# Autodesk Inventor assembly: Ensamblaje1
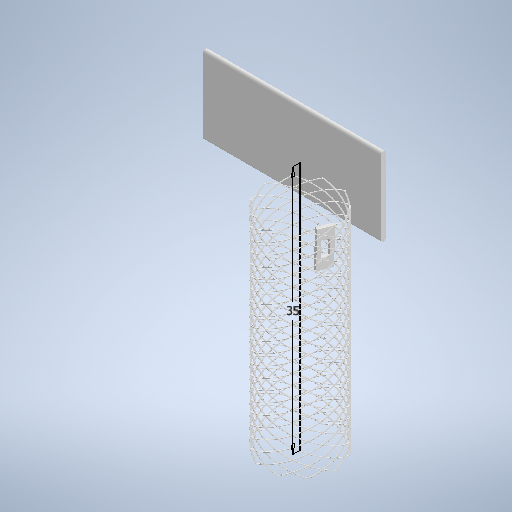
[picture p0: Inventor's stored thumbnail of the model, 512x512]
Saved by Autodesk Inventor 2025.2 (Build 292293000, 293)
## iProperties
Created: 2025-03-06
Part Number: Ensamblaje1
Document SubType Name: Assembly
Designer: julia
Author: julia
## Documents named in this file (4)
- C:\Users\julia\Desktop\ING_SALUD\TFG\Ensamblaje1.iam
- C:\Users\julia\Desktop\ING_SALUD\TFG\stent 1.ipt
- C:\Users\julia\Desktop\ING_SALUD\TFG\placa de amarre.ipt
- C:\Users\julia\Desktop\ING_SALUD\TFG\sensor.ipt
## Components (4 placed, 3 different names)
1. stent 1:1 — Coincidencia:1, Coincidencia:2
2. placa de amarre:1 — Coincidencia:1, Coincidencia:2
3. sensor:1 — Coincidencia:3, Coincidencia:4
4. placa de amarre:2 — Coincidencia:3, Coincidencia:4
## Relationships (4: Mate 4)
- Coincidencia:1 [Mate]: stent 1:1 ↔ placa de amarre:1
- Coincidencia:2 [Mate]: stent 1:1 ↔ placa de amarre:1
- Coincidencia:3 [Mate]: sensor:1 ↔ placa de amarre:2
- Coincidencia:4 [Mate]: sensor:1 ↔ placa de amarre:2
